# Autodesk Inventor assembly: Motor_assembly
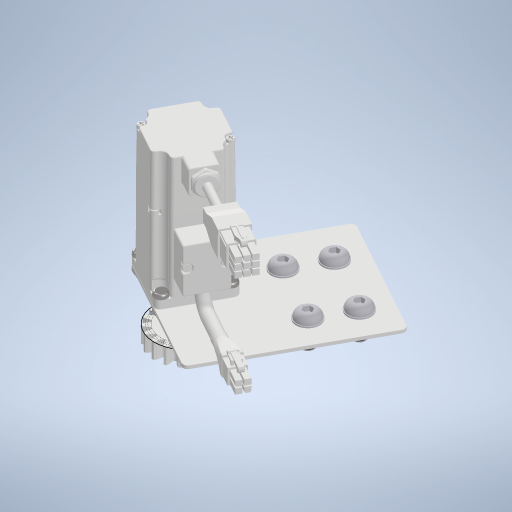
[picture p0: Inventor's stored thumbnail of the model, 512x512]
Saved by Autodesk Inventor 2023 (Build 270158000, 158)
## iProperties
Created: 2022-08-24
Part Number: Motor_assembly
Document SubType Name: Assembly
Designer: matte
Author: matte
## Documents named in this file (9)
- C:\Users\matte\Documents\GitHub\MDM-CyberOrto-CAD\Rack_Pinion\Motor_assembly.iam
- C:\Users\matte\Documents\GitHub\MDM-CyberOrto-CAD\Rack_Pinion\piastra_motore.ipt
- C:\Users\matte\Documents\GitHub\MDM-CyberOrto-CAD\Servo Motor 50W\bch2mba531ca5c.ipt
- C:\Users\matte\Documents\GitHub\MDM-CyberOrto-CAD\Inventor Support\Content Center Files\it-IT\AS 1474(1)\AS 1474 - M4(1).ipt
- C:\Users\matte\Documents\GitHub\MDM-CyberOrto-CAD\Inventor Support\Content Center Files\it-IT\ISO 1580\ISO 1580 - M4 x 12_.ipt
- C:\Users\matte\Documents\GitHub\MDM-CyberOrto-CAD\Parker components\02-Fasteners\10-Standard T-Nuts\20-049.ipt
- C:\Users\matte\Documents\GitHub\MDM-CyberOrto-CAD\Parker components\02-Fasteners\15-T-Bolts_Nuts_Washers\03-Washers\24-708-8.ipt
- C:\Users\matte\Documents\GitHub\MDM-CyberOrto-CAD\Parker components\02-Fasteners\16-Screws\01-Metric Screws\01-Button Head\24-116-8.ipt
- C:\Users\matte\Documents\GitHub\MDM-CyberOrto-CAD\Rack_Pinion\Pinion.ipt
## Components (21 placed, 8 different names)
1. piastra_motore:1 — Coincidente:2, Coincidente:3, Coincidente:5, Coincidente:6, Coincidente:7, Allineato:3, Coincidente:8, Coincidente:9, Allineato:7, Allineato:8
2. bch2mba531ca5c:1 — Coincidente:2, Coincidente:4, Allineato:7, Allineato:8, Coincidente:12, Angolo:1, Coincidente:13
3. 20-049:1 — Coincidente:6, Coincidente:7, Allineato:3, Allineato:4, Allineato:5, Allineato:6
4. 20-049:2 — Allineato:4, Allineato:5, Allineato:6
5. Pinion:1 — Coincidente:12, Angolo:1, Coincidente:13
6. AS 1474 - Metrico M4:1 — Coincidente:3
7. ISO 1580 M4 x 12:1 — Coincidente:4, Coincidente:5
8. AS 1474 - Metrico M4:2
9. ISO 1580 M4 x 12:2
10. AS 1474 - Metrico M4:3
11. ISO 1580 M4 x 12:3
12. AS 1474 - Metrico M4:4
13. ISO 1580 M4 x 12:4
14. 24-116-8:1 — Coincidente:10, Coincidente:11
15. 24-708-8:1 — Coincidente:8, Coincidente:9, Coincidente:10, Coincidente:11
16. 24-116-8:2
17. 24-708-8:2
18. 24-116-8:3
19. 24-708-8:3
20. 24-116-8:4
21. 24-708-8:4
## Component patterns: (4 elements, first: AS 1474 - Metrico M4:1 + ISO 1580 M4 x 12:1), (4 elements, first: 24-116-8:1 + 24-708-8:1)
## Relationships (20: Mate 13, Flush 6, Angle 1)
- [Mate]: AS 1474 - Metrico M4:1 ↔ ISO 1580 M4 x 12:1
- Coincidente:2 [Mate]: piastra_motore:1 ↔ bch2mba531ca5c:1
- Coincidente:3 [Mate]: piastra_motore:1 ↔ AS 1474 - Metrico M4:1
- Coincidente:4 [Mate]: bch2mba531ca5c:1 ↔ ISO 1580 M4 x 12:1
- Coincidente:5 [Mate]: piastra_motore:1 ↔ ISO 1580 M4 x 12:1
- Coincidente:6 [Mate] (-20 mm): piastra_motore:1 ↔ 20-049:1
- Coincidente:7 [Mate] (4.5 mm): piastra_motore:1 ↔ 20-049:1
- Allineato:3 [Flush] (10 mm): piastra_motore:1 ↔ 20-049:1
- Allineato:4 [Flush]: 20-049:1 ↔ 20-049:2
- Allineato:5 [Flush]: 20-049:1 ↔ 20-049:2
- Allineato:6 [Flush] (-40 mm): 20-049:1 ↔ 20-049:2
- Coincidente:8 [Mate]: piastra_motore:1 ↔ 24-708-8:1
- Coincidente:9 [Mate]: piastra_motore:1 ↔ 24-708-8:1
- Coincidente:10 [Mate]: 24-116-8:1 ↔ 24-708-8:1
- Coincidente:11 [Mate]: 24-116-8:1 ↔ 24-708-8:1
- Allineato:7 [Flush]: piastra_motore:1 ↔ bch2mba531ca5c:1
- Allineato:8 [Flush]: piastra_motore:1 ↔ bch2mba531ca5c:1
- Coincidente:12 [Mate]: bch2mba531ca5c:1 ↔ Pinion:1
- Angolo:1 [Angle] (180 deg): bch2mba531ca5c:1 ↔ Pinion:1
- Coincidente:13 [Mate]: bch2mba531ca5c:1 ↔ Pinion:1
## Named parameters: d78_d351 = 0 mm
